# Autodesk Inventor assembly: Bearing Flat NScrew Slotted Right
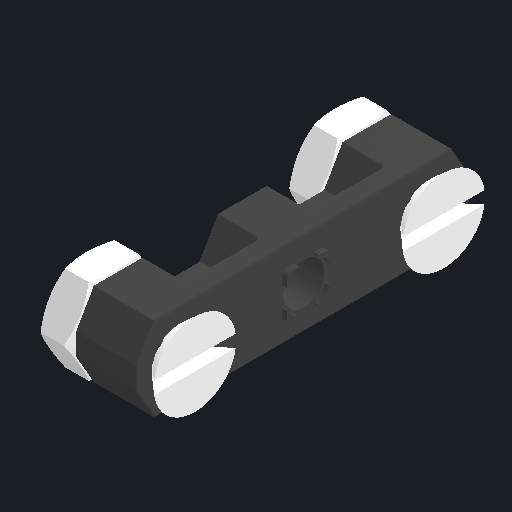
[picture p0: Inventor's stored thumbnail of the model, 512x512]
Saved by Autodesk Inventor 2025 (Build 290162000, 162)
## iProperties
Created: 2024-10-10
Part Number: Bearing Flat NScrew Slotted Right
Document SubType Name: Assembly
Designer: Averey Ku
Author: Averey Ku
## Documents named in this file (5)
- D:\VEX\High Stakes\CAD\V2\Chassis\Drivebay Right\Bearing Flat NScrew Slotted Right.iam
- D:\VEX\High Stakes\CAD\V2\Chassis\Drivebay Right\NScrew Slotted Threaded .500 Right.ipt
- D:\VEX\High Stakes\CAD\V2\Chassis\Drivebay Right\Bearing Flat Low Profile Right.ipt
- D:\VEX\High Stakes\CAD\ROBOPROS-CAD-Inventor\Structure\Hardware\Nut Nylon\Nut Nylon - White.ipt
- D:\VEX\High Stakes\CAD\ROBOPROS-CAD-Inventor\Structure\Hardware\Nut Nylon.ipt
## Components (7 placed, 3 different names)
1. NScrew Slotted Threaded .500 Right:1 — Insert:1
2. NScrew Slotted Threaded .500 Right:2 — Insert:2
3. Bearing Flat Low Profile Right:1 — Insert:2, Insert:1, Insert:4, Insert:3, Insert:6, Insert:5
4. Nut Nylon - White:1 — Insert:4
5. Nut Nylon - White:2 — Insert:3
6. NScrew Slotted Threaded .500 Right:3 — Insert:6
7. NScrew Slotted Threaded .500 Right:4 — Insert:5
## Relationships (6: Insert 6)
- Insert:2 (-3.175 mm): NScrew Slotted Threaded .500 Right:2 ↔ Bearing Flat Low Profile Right:1
- Insert:1 (-3.175 mm): NScrew Slotted Threaded .500 Right:1 ↔ Bearing Flat Low Profile Right:1
- Insert:4 (1.27 mm): Bearing Flat Low Profile Right:1 ↔ Nut Nylon - White:1
- Insert:3 (1.27 mm): Bearing Flat Low Profile Right:1 ↔ Nut Nylon - White:2
- Insert:6 (-1.5875 mm): Bearing Flat Low Profile Right:1 ↔ NScrew Slotted Threaded .500 Right:3
- Insert:5 (-1.5875 mm): Bearing Flat Low Profile Right:1 ↔ NScrew Slotted Threaded .500 Right:4
